# Autodesk Inventor assembly: Assembly1
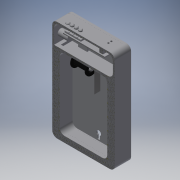
[picture p0: Inventor's stored thumbnail of the model, 180x180]
Saved by Autodesk Inventor 2019 (Build 230136000, 136)
## iProperties
Created: 2020-07-16
Part Number: Assembly1
Document SubType Name: Assembly
Designer: Erle
Author: Erle
## Documents named in this file (12)
- C:\Users\Erle\Desktop\Slow Motion\SloMo\Assembly1.iam
- C:\Users\Erle\Desktop\Slow Motion\SloMo\Bottom.ipt
- C:\Users\Erle\Desktop\Slow Motion\SloMo\Test2.ipt
- C:\Users\Erle\Desktop\Slow Motion\SloMo\Feder.ipt
- C:\Users\Erle\Desktop\Slow Motion\SloMo\Magnet.ipt
- C:\Users\Erle\Desktop\Slow Motion\SloMo\din1587-m4x0_76.ipt
- C:\Users\Erle\Desktop\Slow Motion\SloMo\Insert.ipt
- C:\Users\Erle\Desktop\Slow Motion\SloMo\Platine.ipt
- C:\Users\Erle\Desktop\Slow Motion\SloMo\Knopf.ipt
- C:\Users\Erle\Desktop\Slow Motion\SloMo\Strom.ipt
- C:\Users\Erle\Desktop\Slow Motion\SloMo\din_912-m4x0_7-20-8_8.ipt
- C:\Users\Erle\Desktop\Slow Motion\SloMo\Top.ipt
## Components (18 placed, 11 different names)
1. Bottom:1 — Mate:1, Mate:2, Flush:1, Mate:4, Mate:5, Mate:6, Mate:7, Mate:8, Mate:9, Mate:10, Mate:11, Mate:12, Flush:4, Flush:5, Flush:6, Flush:7, Mate:13, Mate:14, Mate:15, Mate:16, Mate:17, Mate:18, Mate:19, Mate:20, Mate:22, Mate:27, Mate:28, Mate:29
2. Test2:1 — Mate:3, Flush:2, Flush:3, Mate:4, Mate:21, Mate:22, Mate:23, Mate:24, Mate:25
3. Test2:2 — Mate:3, Flush:2, Flush:3, Mate:5
4. Feder:1 — Mate:6, Mate:7, Mate:8, Mate:26
5. Magnet:1 — Mate:26
6. din1587-m4x0_76:1 — Mate:21, Mate:23
7. Insert:1 — Mate:12, Flush:4
8. Insert:2 — Mate:11, Flush:5
9. Insert:3 — Mate:9, Flush:7
10. Insert:4 — Mate:10, Flush:6
11. Platine:1 — Mate:13, Mate:14
12. Knopf:1 — Mate:18
13. Knopf:2 — Mate:17
14. Knopf:3 — Mate:16
15. Knopf:4 — Mate:15
16. Strom:1 — Mate:19, Mate:20
17. din_912-m4x0_7-20-8_8:1 — Mate:24, Mate:25
18. Top:1 — Mate:27, Mate:28, Mate:29
## Relationships (36: Mate 29, Flush 7)
- Mate:1: Bottom:1
- Mate:2: Bottom:1
- Flush:1: Bottom:1
- Mate:3: Test2:1 ↔ Test2:2
- Flush:2: Test2:1 ↔ Test2:2
- Flush:3: Test2:1 ↔ Test2:2
- Mate:4: Bottom:1 ↔ Test2:1
- Mate:5: Bottom:1 ↔ Test2:2
- Mate:6: Bottom:1 ↔ Feder:1
- Mate:7: Bottom:1 ↔ Feder:1
- Mate:8: Bottom:1 ↔ Feder:1
- Mate:9: Bottom:1 ↔ Insert:3
- Mate:10: Bottom:1 ↔ Insert:4
- Mate:11: Bottom:1 ↔ Insert:2
- Mate:12: Bottom:1 ↔ Insert:1
- Flush:4: Bottom:1 ↔ Insert:1
- Flush:5: Bottom:1 ↔ Insert:2
- Flush:6: Bottom:1 ↔ Insert:4
- Flush:7: Bottom:1 ↔ Insert:3
- Mate:13: Bottom:1 ↔ Platine:1
- Mate:14: Bottom:1 ↔ Platine:1
- Mate:15: Bottom:1 ↔ Knopf:4
- Mate:16: Bottom:1 ↔ Knopf:3
- Mate:17: Bottom:1 ↔ Knopf:2
- Mate:18: Bottom:1 ↔ Knopf:1
- Mate:19: Bottom:1 ↔ Strom:1
- Mate:20: Bottom:1 ↔ Strom:1
- Mate:21: Test2:1 ↔ din1587-m4x0_76:1
- Mate:22: Bottom:1 ↔ Test2:1
- Mate:23: Test2:1 ↔ din1587-m4x0_76:1
- Mate:24: Test2:1 ↔ din_912-m4x0_7-20-8_8:1
- Mate:25: Test2:1 ↔ din_912-m4x0_7-20-8_8:1
- Mate:26: Feder:1 ↔ Magnet:1
- Mate:27: Bottom:1 ↔ Top:1
- Mate:28 (0.5 mm): Bottom:1 ↔ Top:1
- Mate:29 (0.5 mm): Bottom:1 ↔ Top:1
